# Autodesk Inventor assembly: ASM_Micron_ASAP_Merge_v3_rendering
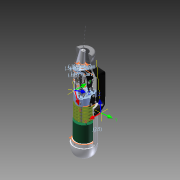
[picture p0: Inventor's stored thumbnail of the model, 180x180]
Saved by Autodesk Inventor 2011 SP2 (Build 150309200, 309)
## iProperties
Created: 2011-10-07
Part Number: ASM_Micron_ASAP_Merge_v3_rendering
Document SubType Name: Assembly
Designer: sungwook
Author: sungwook
## Documents named in this file (31)
- C:\Users\sungwook\Documents\Inventor\Micron20_Base_Tube_Adjst\Assembly\Motion_Merge\ASM_Micron_ASAP_Merge_v3_rendering.iam
- C:\Users\sungwook\Documents\Inventor\Micron20_Base_Tube_Adjst\Assembly\Motion_Merge\Indep\ASM_Micron_ASAP_Indep0.iam
- C:\Users\sungwook\Documents\Inventor\Micron20_Base_Tube_Adjst\Assembly\Motion_Merge\Indep\ASM_Micron_ASAP_Indep10.iam
- C:\Users\sungwook\Documents\Inventor\Micron20_Base_Tube_Adjst\Assembly\Motion_Merge\Indep\ASM_Micron_ASAP_Indep20.iam
- C:\Users\sungwook\Documents\Inventor\Micron20_Base_Tube_Adjst\Assembly\Motion_Merge\Indep\ASM_Micron_ASAP_Indep30.iam
- C:\Users\sungwook\Documents\Inventor\Micron20_Base_Tube_Adjst\Assembly\Motion_Merge\Indep\ASM_Micron_ASAP_Indep40.iam
- C:\Users\sungwook\Documents\Inventor\Micron20_Base_Tube_Adjst\Assembly\Motion_Merge\Indep\ASM_Micron_ASAP_Indep50.iam
- C:\Users\sungwook\Documents\Inventor\Micron20_Base_Tube_Adjst\Assembly\Motion_Merge\Indep\ASM_Micron_ASAP_Indep60.iam
- C:\Users\sungwook\Documents\Inventor\Micron20_Base_Tube_Adjst\Assembly\Motion_Merge\Indep\ASM_Micron_ASAP_Indep70.iam
- C:\Users\sungwook\Documents\Inventor\Micron20_Base_Tube_Adjst\Assembly\Motion_Merge\Indep\ASM_Micron_ASAP_Indep80.iam
- C:\Users\sungwook\Documents\Inventor\Micron20_Base_Tube_Adjst\Assembly\Motion_Merge\Indep\ASM_Micron_ASAP_Indep90.iam
- C:\Users\sungwook\Documents\Inventor\Micron20_Base_Tube_Adjst\Assembly\Motion_Merge\Indep\ASM_Micron_ASAP_Indep100.iam
- C:\Users\sungwook\Documents\Inventor\Micron20_Base_Tube_Adjst\Assembly\Motion_Merge\Indep\ASM_Micron_ASAP_Indep110.iam
- C:\Users\sungwook\Documents\Inventor\Micron20_Base_Tube_Adjst\Assembly\Motion_Merge\Indep\ASM_Micron_ASAP_Indep120.iam
- C:\Users\sungwook\Documents\Inventor\Micron20_Base_Tube_Adjst\Assembly\Motion_Merge\Indep\ASM_Micron_ASAP_Indep130.iam
- C:\Users\sungwook\Documents\Inventor\Micron20_Base_Tube_Adjst\Assembly\Motion_Merge\Indep\ASM_Micron_ASAP_Indep140.iam
- C:\Users\sungwook\Documents\Inventor\Micron20_Base_Tube_Adjst\Parts\ASAP\Handle_ASAP.iam
- C:\Users\sungwook\Documents\Inventor\Micron20_Base_Tube_Adjst\Parts\Electronics\PCB_Stack.iam
- C:\Users\sungwook\Documents\Inventor\Micron20_Base_Tube_Adjst\Parts\Handle\Handle_1_rev.ipt
- C:\Users\sungwook\Documents\Inventor\Micron20_Base_Tube_Adjst\Parts\Handle\Ver1(RP)\part\Handle_1_rev_Back.ipt
- C:\Users\sungwook\Documents\Inventor\Micron20_Base_Tube_Adjst\Parts\Handle\Ver1(RP)\Handle_1_rev_Back_part1.ipt
- C:\Users\sungwook\Documents\Inventor\Micron20_Base_Tube_Adjst\Parts\Handle\Ver1(RP)\Handle_1_rev_Back_part2.ipt
- C:\Users\sungwook\Documents\Inventor\Micron20_Base_Tube_Adjst\Parts\Handle\Window.ipt
- C:\Users\sungwook\Documents\Inventor\Micron20_Base_Tube_Adjst\Parts\Handle\Ver2(Al_RP)\Handle_2_Asm.iam
- C:\Users\sungwook\Documents\Inventor\Micron20_Base_Tube_Adjst\06082012_Outer_Tube\Outer_Tube.ipt
- C:\Users\sungwook\Documents\Inventor\Content Center Files\R2011\en-US\ANSI B18.6.3(00)\ANSI B18.6.3 - 0-80 UNF - 0.1875(32).ipt
- C:\Users\sungwook\Documents\Inventor\Micron20_Base_Tube_Adjst\Parts\Handle\Ver2(Al_RP)\Handle_2_Back_rev2.ipt
- C:\Users\sungwook\Documents\Inventor\Micron20_Base_Tube_Adjst\04192012_New_Front_2pcs\New_Front_Base_rev.ipt
- C:\Users\sungwook\Documents\Inventor\Micron20_Base_Tube_Adjst\04192012_New_Front_2pcs\New_Front_Upper_rev.ipt
- C:\Users\sungwook\Documents\Inventor\Micron20_Base_Tube_Adjst\04192012_New_Front_2pcs\New_Front_Upper_rev_v2.ipt
- C:\Users\sungwook\Documents\Inventor\Micron20_Base_Tube_Adjst\04192012_New_Front_2pcs\New_Front_Upper_rev_v3.ipt
## Components (32 placed, 30 different names)
1. (0,0,0) [sub-assembly] — Flush:2, Mate:2, Flush:4, Flush:6, Flush:8, Flush:10, Flush:12, Flush:14, Flush:16, Flush:18, Flush:21, Flush:24, Flush:26, Flush:28, Mate:28, Mate:29, Mate:30, Mate:31, Mate:32, Mate:33, Mate:34, Mate:35, Mate:36, Mate:37, Mate:38, Mate:39, Mate:40, Mate:41, Mate:42, Mate:43, Mate:44, Mate:45, Mate:46, Mate:47, Mate:48, Mate:49, Mate:50, Flush:31, Mate:51, Mate:52, Mate:53, Mate:54, Mate:55, Mate:73, Mate:74, Mate:94, Mate:107, Mate:108
2. (0,2,0) [sub-assembly] — Flush:2, Mate:28, Mate:29
3. pi/2,2,0 [sub-assembly] — Flush:4, Flush:30, Mate:30
4. pi,2,0 [sub-assembly] — Flush:6, Mate:31, Mate:32
5. -pi/2,2,0 [sub-assembly] — Flush:8, Mate:33, Mate:34
6. 0,0,-2 [sub-assembly] — Flush:10, Mate:37, Mate:38
7. 0,2,-2 [sub-assembly] — Flush:12, Mate:39, Mate:40
8. pi/2,2,-2 [sub-assembly] — Flush:21, Mate:41, Mate:42
9. pi,2,-2 [sub-assembly] — Flush:16, Mate:35, Mate:36
10. -pi/2,2,-2 [sub-assembly] — Flush:14, Mate:43, Mate:44
11. 0,0,2 [sub-assembly] — Flush:18, Mate:45, Mate:46
12. 0,2,2 [sub-assembly] — Flush:28, Mate:47, Mate:48
13. pi/2,2,2 [sub-assembly] — Mate:49, Mate:50, Flush:31
14. pi,2,2 [sub-assembly] — Flush:24, Mate:51, Mate:52
15. -pi/2,2,2 [sub-assembly] — Flush:26, Mate:53, Mate:54, Mate:56, Mate:72
16. Handle_ASAP:1 [sub-assembly] — Mate:55, Mate:56
17. PCB_Stack:1 [sub-assembly] — Mate:72, Flush:73, Mate:73, Mate:74, Mate:103
18. Window:1
19. Handle_1_rev_total — Mate:77, Mate:78
20. Handle_1_rev_Back:1
21. Handle_1_rev_Back_part1:1 — Mate:93, Mate:96
22. Handle_1_rev_Back_part2:1 — Mate:93, Mate:94, Mate:96
23. Handle_2_Asm:1 [sub-assembly] — Mate:101, Mate:102, Mate:103
24. New_Front_Base_rev:1 — Mate:112, Mate:113, Mate:114, Flush:74, Mate:120, Flush:121, Mate:121, Flush:123
25. New_Front_Upper_rev:1 — Mate:117, Flush:74, Mate:118, Mate:119
26. New_Front_Upper_rev_v2:1 — Mate:120, Flush:121, Flush:122
27. New_Front_Upper_rev_v3:1 — Mate:121, Flush:123, Flush:124
28. Handle_2_Back_rev2:1 — Mate:109, Mate:110, Mate:111
29. Outer_Tube:1 — Mate:104, Mate:105, Mate:108, Mate:109, Mate:111, Mate:114, Mate:117, Mate:118, Mate:119, Flush:122, Flush:124
30. Cross Recessed 100° Flat Countersunk Head Machine Screw - Type I - Inch 0-80 UNF x 0.1875:1 — Mate:107
31. Cross Recessed 100° Flat Countersunk Head Machine Screw - Type I - Inch 0-80 UNF x 0.1875:2
32. Cross Recessed 100° Flat Countersunk Head Machine Screw - Type I - Inch 0-80 UNF x 0.1875:3
## Component patterns: (3 elements, first: Cross Recessed 100° Flat Countersunk Head Machine Screw - Type I - Inch 0-80 UNF x 0.1875:1)
## Relationships (77: Mate 56, Flush 21)
- Flush:2: (0,0,0) ↔ (0,2,0)
- Mate:2: (0,0,0)
- Flush:4: (0,0,0) ↔ pi/2,2,0
- Flush:6: (0,0,0) ↔ pi,2,0
- Flush:8: (0,0,0) ↔ -pi/2,2,0
- Flush:10: (0,0,0) ↔ 0,0,-2
- Flush:12: (0,0,0) ↔ 0,2,-2
- Flush:14: (0,0,0) ↔ -pi/2,2,-2
- Flush:16: (0,0,0) ↔ pi,2,-2
- Flush:18: (0,0,0) ↔ 0,0,2
- Flush:21: (0,0,0) ↔ pi/2,2,-2
- Flush:24: (0,0,0) ↔ pi,2,2
- Flush:26: (0,0,0) ↔ -pi/2,2,2
- Flush:28: (0,0,0) ↔ 0,2,2
- Mate:28: (0,0,0) ↔ (0,2,0)
- Mate:29: (0,0,0) ↔ (0,2,0)
- Flush:30: pi/2,2,0
- Mate:30: (0,0,0) ↔ pi/2,2,0
- Mate:31: (0,0,0) ↔ pi,2,0
- Mate:32: (0,0,0) ↔ pi,2,0
- Mate:33: (0,0,0) ↔ -pi/2,2,0
- Mate:34: (0,0,0) ↔ -pi/2,2,0
- Mate:35: (0,0,0) ↔ pi,2,-2
- Mate:36: (0,0,0) ↔ pi,2,-2
- Mate:37: (0,0,0) ↔ 0,0,-2
- Mate:38: (0,0,0) ↔ 0,0,-2
- Mate:39: (0,0,0) ↔ 0,2,-2
- Mate:40: (0,0,0) ↔ 0,2,-2
- Mate:41: (0,0,0) ↔ pi/2,2,-2
- Mate:42: (0,0,0) ↔ pi/2,2,-2
- Mate:43: (0,0,0) ↔ -pi/2,2,-2
- Mate:44: (0,0,0) ↔ -pi/2,2,-2
- Mate:45: (0,0,0) ↔ 0,0,2
- Mate:46: (0,0,0) ↔ 0,0,2
- Mate:47: (0,0,0) ↔ 0,2,2
- Mate:48: (0,0,0) ↔ 0,2,2
- Mate:49: (0,0,0) ↔ pi/2,2,2
- Mate:50: (0,0,0) ↔ pi/2,2,2
- Flush:31: (0,0,0) ↔ pi/2,2,2
- Mate:51: (0,0,0) ↔ pi,2,2
- Mate:52: (0,0,0) ↔ pi,2,2
- Mate:53: (0,0,0) ↔ -pi/2,2,2
- Mate:54: (0,0,0) ↔ -pi/2,2,2
- Mate:55: (0,0,0) ↔ Handle_ASAP:1
- Mate:56: -pi/2,2,2 ↔ Handle_ASAP:1
- Mate:72: -pi/2,2,2 ↔ PCB_Stack:1
- Flush:73: PCB_Stack:1
- Mate:73: (0,0,0) ↔ PCB_Stack:1
- Mate:74: (0,0,0) ↔ PCB_Stack:1
- Mate:77: Handle_1_rev_total
- Mate:78: Handle_1_rev_total
- Mate:93: Handle_1_rev_Back_part1:1 ↔ Handle_1_rev_Back_part2:1
- Mate:94: (0,0,0) ↔ Handle_1_rev_Back_part2:1
- Mate:96: Handle_1_rev_Back_part1:1 ↔ Handle_1_rev_Back_part2:1
- Mate:101: Handle_2_Asm:1
- Mate:102: Handle_2_Asm:1
- Mate:103: PCB_Stack:1 ↔ Handle_2_Asm:1
- Mate:104: Outer_Tube:1
- Mate:105: Outer_Tube:1
- Mate:108: (0,0,0) ↔ Outer_Tube:1
- Mate:109: Handle_2_Back_rev2:1 ↔ Outer_Tube:1
- Mate:110: Handle_2_Back_rev2:1
- Mate:111: Handle_2_Back_rev2:1 ↔ Outer_Tube:1
- Mate:112: New_Front_Base_rev:1
- Mate:113: New_Front_Base_rev:1
- Mate:114: New_Front_Base_rev:1 ↔ Outer_Tube:1
- Mate:117: New_Front_Upper_rev:1 ↔ Outer_Tube:1
- Flush:74: New_Front_Base_rev:1 ↔ New_Front_Upper_rev:1
- Mate:118: New_Front_Upper_rev:1 ↔ Outer_Tube:1
- Mate:119: New_Front_Upper_rev:1 ↔ Outer_Tube:1
- Mate:120: New_Front_Base_rev:1 ↔ New_Front_Upper_rev_v2:1
- Flush:121: New_Front_Base_rev:1 ↔ New_Front_Upper_rev_v2:1
- Flush:122: New_Front_Upper_rev_v2:1 ↔ Outer_Tube:1
- Mate:121: New_Front_Base_rev:1 ↔ New_Front_Upper_rev_v3:1
- Flush:123: New_Front_Base_rev:1 ↔ New_Front_Upper_rev_v3:1
- Flush:124: New_Front_Upper_rev_v3:1 ↔ Outer_Tube:1
- Mate:107: (0,0,0) ↔ Cross Recessed 100° Flat Countersunk Head Machine Screw - Type I - Inch 0-80 UNF x 0.1875:1
